# Autodesk Inventor assembly: assembly
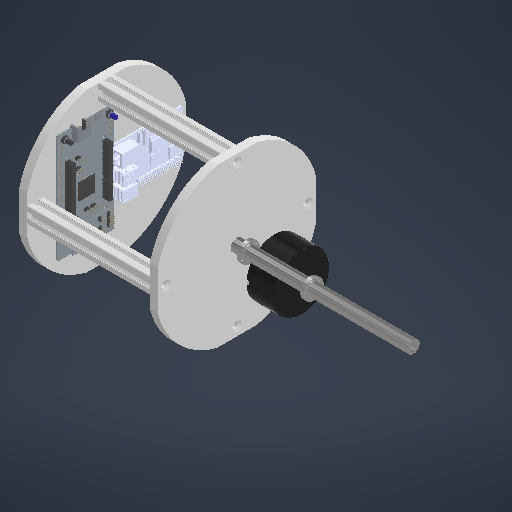
[picture p0: Inventor's stored thumbnail of the model, 512x512]
Saved by Autodesk Inventor 2027 (Build 310192000, 192)
## iProperties
Created: 2026-10-07
Part Number: assembly
Document SubType Name: Assembly
Designer: luca
Author: luca
## Documents named in this file (10)
- C:\Users\luca\Desktop\double_pendulum\RL-Rotary-Inverted-Double-Pendulum\CAD\assembly.iam
- C:\Users\luca\Desktop\double_pendulum\RL-Rotary-Inverted-Double-Pendulum\CAD\motor\L-7015-251029\2D3D\RMD-7015三维图\RMD-7015\RMD-7015.ipt
- C:\Users\luca\Desktop\double_pendulum\RL-Rotary-Inverted-Double-Pendulum\CAD\encoder\AMT102-D2048-I6350-S\3D\AMT102-D2048-I6350-S\AMT102-D2048-I6350-S.ipt
- C:\Users\luca\Desktop\double_pendulum\RL-Rotary-Inverted-Double-Pendulum\CAD\Electronics\RASPBERRY_PI_5\RASPBERRY_PI_5.ipt
- C:\Users\luca\Desktop\double_pendulum\RL-Rotary-Inverted-Double-Pendulum\CAD\Electronics\stm32\NUCLEO-F429ZI--3DModel-STEP-56544\NUCLEO-F429ZI--3DModel-STEP-56544.ipt
- C:\Users\luca\Desktop\double_pendulum\RL-Rotary-Inverted-Double-Pendulum\CAD\al-profil-20x20-drazka-6\al-profil-20x20-drazka-6.ipt
- C:\Users\luca\Desktop\double_pendulum\RL-Rotary-Inverted-Double-Pendulum\CAD\plate_lower.ipt
- C:\Users\luca\Desktop\double_pendulum\RL-Rotary-Inverted-Double-Pendulum\CAD\plate_middle.ipt
- C:\Users\luca\Documents\drive_shaft_center.ipt
- C:\Users\luca\Documents\Inventor\Content Center Files\R2027\de-DE\BS 290 SKF(30)\BS 290 SKF - SKF 61802.ipt
## Components (13 placed, 9 different names)
1. RMD-7015:1 — Passend:11
2. AMT102-D2048-I6350-S:1 — Passend:12, Passend:13
3. RASPBERRY_PI_5:1 — Passend:7
4. NUCLEO-F429ZI--3DModel-STEP-56544:1 — Passend:6
5. plate_lower:1 — Passend:1, Passend:2, Passend:3, Passend:4, Passend:5, Winkel:1, Passend:6, Passend:7
6. plate_middle:1 — Passend:8, Passend:9, Passend:10, Passend:11, Passend:12, Passend:13, Passend:15
7. drive_shaft_center:1 — Passend:14, Passend:15, Passend:16
8. BS 290 SKF 61802:1 — Passend:14
9. BS 290 SKF 61802:2 — Passend:16
10. al-profil-20x20-drazka-6:1 — Passend:4, Passend:5, Winkel:1, Passend:8, Passend:10
11. al-profil-20x20-drazka-6:2 — Passend:9
12. al-profil-20x20-drazka-6:3
13. al-profil-20x20-drazka-6:4
## Component patterns: (4 elements, first: al-profil-20x20-drazka-6:1)
## Relationships (17: Mate 16, Angle 1)
- Passend:1 [Mate]: plate_lower:1
- Passend:2 [Mate]: plate_lower:1
- Passend:3 [Mate]: plate_lower:1
- Passend:4 [Mate]: plate_lower:1 ↔ al-profil-20x20-drazka-6:1
- Passend:5 [Mate]: plate_lower:1 ↔ al-profil-20x20-drazka-6:1
- Winkel:1 [Angle] (0 deg): plate_lower:1 ↔ al-profil-20x20-drazka-6:1
- Passend:6 [Mate]: NUCLEO-F429ZI--3DModel-STEP-56544:1 ↔ plate_lower:1
- Passend:7 [Mate]: RASPBERRY_PI_5:1 ↔ plate_lower:1
- Passend:8 [Mate]: plate_middle:1 ↔ al-profil-20x20-drazka-6:1
- Passend:9 [Mate]: plate_middle:1 ↔ al-profil-20x20-drazka-6:2
- Passend:10 [Mate]: plate_middle:1 ↔ al-profil-20x20-drazka-6:1
- Passend:11 [Mate]: RMD-7015:1 ↔ plate_middle:1
- Passend:12 [Mate]: AMT102-D2048-I6350-S:1 ↔ plate_middle:1
- Passend:13 [Mate]: AMT102-D2048-I6350-S:1 ↔ plate_middle:1
- Passend:14 [Mate]: drive_shaft_center:1 ↔ BS 290 SKF 61802:1
- Passend:15 [Mate]: plate_middle:1 ↔ drive_shaft_center:1
- Passend:16 [Mate]: drive_shaft_center:1 ↔ BS 290 SKF 61802:2
